# Autodesk Inventor assembly: TEST-MODULE-CONJUNTO
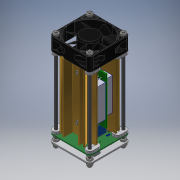
[picture p0: Inventor's stored thumbnail of the model, 180x180]
Saved by Autodesk Inventor 2018.3 (Build 223284000, 284)
## iProperties
Created: 2021-05-04
Part Number: TEST-MODULE-CONJUNTO
Document SubType Name: Assembly
Designer: laguerre
AI: -
B: -
BO: -
BOB: -
BR: -
CCB: -
CCC: -
CO: -
COB: -
COC: -
CR: -
CRB: -
DES: -
GL: -
GLO: -
LA: -
LC: -
LG: -
LGO: -
Linea: -
LT: -
LTC: -
LTO: -
Maquina: -
N: -
NG: -
OBR: -
OBR1: -
OOB: -
OR: -
PC: -
PE: -
PL: -
PO: -
POP: -
QL: -
QLC: -
QLO: -
QR: -
QS: -
QSC: -
QSO: -
RPC: -
RU: -
Sector: -
SG: -
SGO: -
ST: -
STC: -
STO: -
Author: laguerre
## Documents named in this file (13)
- C:\Proyectos\BURN-IN-TEST\TEST-MODULE\3D\TEST-MODULE-CONJUNTO.iam
- C:\Proyectos\BURN-IN-TEST\TEST-MODULE\3D\RESISTOR-BOARD\RESISTORS-BOARD.iam
- C:\Proyectos\BURN-IN-TEST\TEST-MODULE\3D\CF-TOR-0001.ipt
- C:\Proyectos\BURN-IN-TEST\TEST-MODULE\3D\CF-TCA-0001.ipt
- C:\Proyectos\BURN-IN-TEST\TEST-MODULE\3D\PP-LAS-0001.ipt
- C:\Proyectos\BURN-IN-TEST\TEST-MODULE\3D\TEST-MODULE\TEST-MODULE-V2.iam
- C:\Proyectos\BURN-IN-TEST\TEST-MODULE\3D\CF-VAR-0001.ipt
- C:\Proyectos\BURN-IN-TEST\TEST-MODULE\3D\PP-I3D-0001.ipt
- C:\Proyectos\BURN-IN-TEST\TEST-MODULE\3D\CE-ACC-0001.ipt
- C:\Proyectos\BURN-IN-TEST\TEST-MODULE\3D\CF-TCA-0002.ipt
- C:\Proyectos\BURN-IN-TEST\TEST-MODULE\3D\CF-TCA-0003.ipt
- C:\Proyectos\BURN-IN-TEST\TEST-MODULE\3D\CE-VAR-0001.ipt
- C:\Proyectos\BURN-IN-TEST\TEST-MODULE\3D\CF-TOR-0002.ipt
## Components (42 placed, 13 different names)
1. CE-ACC-0001:1 — Coincidencia:10, Coincidencia:11, Coincidencia:13, Ángulo:2, Insertar:1, Insertar:2, Coincidencia:43, Coincidencia:44, Coincidencia:45
2. CE-ACC-0001:2 — Coincidencia:12, Coincidencia:13, Ángulo:1, Insertar:3, Insertar:4
3. RESISTORS-BOARD:1 [sub-assembly] — Coincidencia:10, Coincidencia:11, Coincidencia:12, Ángulo:1, Ángulo:2, Nivelación:14
4. DIN 912 - reemplazado por DIN EN ISO 4762 M3 x 10:1 — Insertar:1
5. DIN 912 - reemplazado por DIN EN ISO 4762 M3 x 10:2 — Insertar:2
6. TUERCA M3:1 — Insertar:4
7. TUERCA M3:2 — Insertar:3
8. PP-LAS-0001:1 — Coincidencia:14, Nivelación:1, Coincidencia:15, Coincidencia:16, Coincidencia:17, Coincidencia:18, Insertar:21, Insertar:22, Insertar:23, Insertar:24, Insertar:26, Insertar:27, Insertar:28, Insertar:32, Insertar:33, Insertar:34, Insertar:35, Insertar:36
9. CE-VAR-0001:1 — Coincidencia:53, Coincidencia:54, Coincidencia:55, Coincidencia:56, Coincidencia:59, Coincidencia:61, Coincidencia:63, Coincidencia:64, Nivelación:18, Nivelación:19, Coincidencia:65, Nivelación:20, Nivelación:21
10. TEST-MODULE-V2:1 [sub-assembly] — Coincidencia:16, Coincidencia:17, Coincidencia:18, Insertar:25, Insertar:29, Insertar:30, Insertar:31, Nivelación:10, Coincidencia:36, Nivelación:11, Coincidencia:38, Coincidencia:40, Coincidencia:42, Nivelación:13
11. CF-VAR-0001:1 — Nivelación:2, Nivelación:5, Coincidencia:39, Coincidencia:52, Coincidencia:53, Coincidencia:62
12. CF-VAR-0001:2 — Nivelación:3, Coincidencia:28, Coincidencia:41, Coincidencia:56, Coincidencia:57
13. CF-VAR-0001:3 — Nivelación:4, Nivelación:5, Coincidencia:30, Coincidencia:37, Coincidencia:54, Coincidencia:60, Coincidencia:66
14. CF-VAR-0001:4 — Nivelación:3, Nivelación:4, Coincidencia:32, Coincidencia:35, Coincidencia:55, Coincidencia:58
15. DIN 934 - reemplazado por DIN EN 24032/28673/28674 M4:13 — Coincidencia:57, Coincidencia:59
16. DIN 934 - reemplazado por DIN EN 24032/28673/28674 M4:14 — Nivelación:2, Coincidencia:52, Coincidencia:63
17. DIN 934 - reemplazado por DIN EN 24032/28673/28674 M4:15 — Coincidencia:60, Coincidencia:61
18. DIN 934 - reemplazado por DIN EN 24032/28673/28674 M4:16 — Coincidencia:58, Coincidencia:65
19. DIN 934 - reemplazado por DIN EN 24032/28673/28674 M4:17 — Insertar:25
20. DIN 934 - reemplazado por DIN EN 24032/28673/28674 M4:18 — Insertar:26
21. DIN 934 - reemplazado por DIN EN 24032/28673/28674 M4:19 — Insertar:28
22. DIN 934 - reemplazado por DIN EN 24032/28673/28674 M4:20 — Insertar:27
23. DIN 934 - reemplazado por DIN EN 24032/28673/28674 M4:21 — Insertar:32, Coincidencia:66
24. DIN 934 - reemplazado por DIN EN 24032/28673/28674 M4:22 — Insertar:29
25. DIN 934 - reemplazado por DIN EN 24032/28673/28674 M4:23 — Insertar:31
26. DIN 934 - reemplazado por DIN EN 24032/28673/28674 M4:24 — Insertar:30
27. DIN 1587 M4:5 — Insertar:22
28. DIN 1587 M4:6 — Insertar:24
29. DIN 1587 M4:7 — Insertar:23
30. DIN 1587 M4:8 — Insertar:21
31. Soporte-Disipador:1 — Coincidencia:45, Coincidencia:62, Coincidencia:64, Nivelación:15, Nivelación:16, Nivelación:21
32. Soporte-Disipador:2 — Coincidencia:28, Nivelación:16, Nivelación:20
33. Soporte-Disipador:3 — Coincidencia:32, Nivelación:17, Nivelación:19
34. Soporte-Disipador:4 — Coincidencia:30, Nivelación:15, Nivelación:17, Nivelación:18
35. Soporte-Disipador:5 — Coincidencia:39, Coincidencia:40, Coincidencia:43, Coincidencia:44
36. Soporte-Disipador:6 — Coincidencia:41, Coincidencia:42, Nivelación:13
37. Soporte-Disipador:7 — Coincidencia:37, Nivelación:11, Coincidencia:38
38. Soporte-Disipador:8 — Coincidencia:35, Nivelación:10, Coincidencia:36
39. CF-TCA-0001:3 — Insertar:35
40. CF-TCA-0001:4 — Insertar:36
41. ISO 7380-1 M3 x 8:3 — Insertar:34
42. ISO 7380-1 M3 x 8:4 — Insertar:33
## Relationships (76: Mate 38, Insert 20, Flush 16, Angle 2)
- Coincidencia:10 [Mate]: CE-ACC-0001:1 ↔ RESISTORS-BOARD:1
- Coincidencia:11 [Mate]: CE-ACC-0001:1 ↔ RESISTORS-BOARD:1
- Coincidencia:12 [Mate]: CE-ACC-0001:2 ↔ RESISTORS-BOARD:1
- Coincidencia:13 [Mate]: CE-ACC-0001:1 ↔ CE-ACC-0001:2
- Ángulo:1 [Angle] (0 deg): CE-ACC-0001:2 ↔ RESISTORS-BOARD:1
- Ángulo:2 [Angle] (0 deg): CE-ACC-0001:1 ↔ RESISTORS-BOARD:1
- Insertar:1: CE-ACC-0001:1 ↔ DIN 912 - reemplazado por DIN EN ISO 4762 M3 x 10:1
- Insertar:2: CE-ACC-0001:1 ↔ DIN 912 - reemplazado por DIN EN ISO 4762 M3 x 10:2
- Insertar:3: CE-ACC-0001:2 ↔ TUERCA M3:2
- Insertar:4: CE-ACC-0001:2 ↔ TUERCA M3:1
- Coincidencia:14 [Mate]: PP-LAS-0001:1
- Nivelación:1 [Flush]: PP-LAS-0001:1
- Coincidencia:15 [Mate]: PP-LAS-0001:1
- Coincidencia:16 [Mate]: PP-LAS-0001:1 ↔ TEST-MODULE-V2:1
- Coincidencia:17 [Mate]: PP-LAS-0001:1 ↔ TEST-MODULE-V2:1
- Coincidencia:18 [Mate] (9 mm): PP-LAS-0001:1 ↔ TEST-MODULE-V2:1
- Nivelación:2 [Flush] (-2 mm): CF-VAR-0001:1 ↔ DIN 934 - reemplazado por DIN EN 24032/28673/28674 M4:14
- Nivelación:3 [Flush]: CF-VAR-0001:2 ↔ CF-VAR-0001:4
- Nivelación:4 [Flush]: CF-VAR-0001:3 ↔ CF-VAR-0001:4
- Nivelación:5 [Flush]: CF-VAR-0001:1 ↔ CF-VAR-0001:3
- Insertar:21: PP-LAS-0001:1 ↔ DIN 1587 M4:8
- Insertar:22: PP-LAS-0001:1 ↔ DIN 1587 M4:5
- Insertar:23: PP-LAS-0001:1 ↔ DIN 1587 M4:7
- Insertar:24: PP-LAS-0001:1 ↔ DIN 1587 M4:6
- Insertar:25: TEST-MODULE-V2:1 ↔ DIN 934 - reemplazado por DIN EN 24032/28673/28674 M4:17
- Insertar:26: PP-LAS-0001:1 ↔ DIN 934 - reemplazado por DIN EN 24032/28673/28674 M4:18
- Insertar:27: PP-LAS-0001:1 ↔ DIN 934 - reemplazado por DIN EN 24032/28673/28674 M4:20
- Insertar:28: PP-LAS-0001:1 ↔ DIN 934 - reemplazado por DIN EN 24032/28673/28674 M4:19
- Insertar:29: TEST-MODULE-V2:1 ↔ DIN 934 - reemplazado por DIN EN 24032/28673/28674 M4:22
- Insertar:30: TEST-MODULE-V2:1 ↔ DIN 934 - reemplazado por DIN EN 24032/28673/28674 M4:24
- Insertar:31: TEST-MODULE-V2:1 ↔ DIN 934 - reemplazado por DIN EN 24032/28673/28674 M4:23
- Insertar:32: PP-LAS-0001:1 ↔ DIN 934 - reemplazado por DIN EN 24032/28673/28674 M4:21
- Coincidencia:28 [Mate]: CF-VAR-0001:2 ↔ Soporte-Disipador:2
- Coincidencia:30 [Mate]: CF-VAR-0001:3 ↔ Soporte-Disipador:4
- Coincidencia:32 [Mate]: CF-VAR-0001:4 ↔ Soporte-Disipador:3
- Coincidencia:35 [Mate]: CF-VAR-0001:4 ↔ Soporte-Disipador:8
- Nivelación:10 [Flush]: TEST-MODULE-V2:1 ↔ Soporte-Disipador:8
- Coincidencia:36 [Mate]: TEST-MODULE-V2:1 ↔ Soporte-Disipador:8
- Coincidencia:37 [Mate]: CF-VAR-0001:3 ↔ Soporte-Disipador:7
- Nivelación:11 [Flush]: TEST-MODULE-V2:1 ↔ Soporte-Disipador:7
- Coincidencia:38 [Mate]: TEST-MODULE-V2:1 ↔ Soporte-Disipador:7
- Coincidencia:39 [Mate]: CF-VAR-0001:1 ↔ Soporte-Disipador:5
- Coincidencia:40 [Mate]: TEST-MODULE-V2:1 ↔ Soporte-Disipador:5
- Coincidencia:41 [Mate]: CF-VAR-0001:2 ↔ Soporte-Disipador:6
- Coincidencia:42 [Mate]: TEST-MODULE-V2:1 ↔ Soporte-Disipador:6
- Nivelación:13 [Flush]: TEST-MODULE-V2:1 ↔ Soporte-Disipador:6
- Nivelación:14 [Flush]: RESISTORS-BOARD:1
- Coincidencia:43 [Mate]: CE-ACC-0001:1 ↔ Soporte-Disipador:5
- Coincidencia:44 [Mate]: CE-ACC-0001:1 ↔ Soporte-Disipador:5
- Coincidencia:45 [Mate]: CE-ACC-0001:1 ↔ Soporte-Disipador:1
- Insertar:33: PP-LAS-0001:1 ↔ ISO 7380-1 M3 x 8:4
- Insertar:34: PP-LAS-0001:1 ↔ ISO 7380-1 M3 x 8:3
- Coincidencia:52 [Mate]: CF-VAR-0001:1 ↔ DIN 934 - reemplazado por DIN EN 24032/28673/28674 M4:14
- Coincidencia:53 [Mate]: CE-VAR-0001:1 ↔ CF-VAR-0001:1
- Coincidencia:54 [Mate]: CE-VAR-0001:1 ↔ CF-VAR-0001:3
- Coincidencia:55 [Mate]: CE-VAR-0001:1 ↔ CF-VAR-0001:4
- Coincidencia:56 [Mate]: CE-VAR-0001:1 ↔ CF-VAR-0001:2
- Coincidencia:57 [Mate]: CF-VAR-0001:2 ↔ DIN 934 - reemplazado por DIN EN 24032/28673/28674 M4:13
- Coincidencia:58 [Mate]: CF-VAR-0001:4 ↔ DIN 934 - reemplazado por DIN EN 24032/28673/28674 M4:16
- Coincidencia:59 [Mate]: CE-VAR-0001:1 ↔ DIN 934 - reemplazado por DIN EN 24032/28673/28674 M4:13
- Coincidencia:60 [Mate]: CF-VAR-0001:3 ↔ DIN 934 - reemplazado por DIN EN 24032/28673/28674 M4:15
- Coincidencia:61 [Mate]: CE-VAR-0001:1 ↔ DIN 934 - reemplazado por DIN EN 24032/28673/28674 M4:15
- Coincidencia:62 [Mate]: CF-VAR-0001:1 ↔ Soporte-Disipador:1
- Coincidencia:63 [Mate]: CE-VAR-0001:1 ↔ DIN 934 - reemplazado por DIN EN 24032/28673/28674 M4:14
- Coincidencia:64 [Mate]: CE-VAR-0001:1 ↔ Soporte-Disipador:1
- Nivelación:15 [Flush]: Soporte-Disipador:1 ↔ Soporte-Disipador:4
- Nivelación:16 [Flush]: Soporte-Disipador:1 ↔ Soporte-Disipador:2
- Nivelación:17 [Flush]: Soporte-Disipador:3 ↔ Soporte-Disipador:4
- Nivelación:18 [Flush]: CE-VAR-0001:1 ↔ Soporte-Disipador:4
- Nivelación:19 [Flush]: CE-VAR-0001:1 ↔ Soporte-Disipador:3
- Coincidencia:65 [Mate]: CE-VAR-0001:1 ↔ DIN 934 - reemplazado por DIN EN 24032/28673/28674 M4:16
- Nivelación:20 [Flush]: CE-VAR-0001:1 ↔ Soporte-Disipador:2
- Nivelación:21 [Flush]: CE-VAR-0001:1 ↔ Soporte-Disipador:1
- Coincidencia:66 [Mate]: CF-VAR-0001:3 ↔ DIN 934 - reemplazado por DIN EN 24032/28673/28674 M4:21
- Insertar:35: PP-LAS-0001:1 ↔ CF-TCA-0001:3
- Insertar:36: PP-LAS-0001:1 ↔ CF-TCA-0001:4
